# Autodesk Inventor assembly: linac_upper_holder-asm
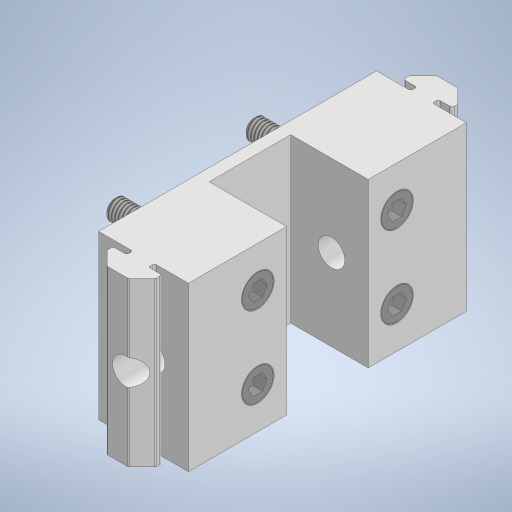
[picture p0: Inventor's stored thumbnail of the model, 512x512]
Saved by Autodesk Inventor 2024 (Build 280153000, 153)
## iProperties
Created: 2025-12-26
Part Number: linac_upper_holder-asm
Document SubType Name: Assembly
Designer: schar
Author: schar
## Documents named in this file (3)
- C:\Users\schar\Desktop\projectBlueprint\AMSTS\hardware\linac_upper_holder-asm.iam
- C:\Users\schar\Desktop\projectBlueprint\AMSTS\hardware\linac_upper_holder.ipt
- C:\Users\schar\Documents\Inventor\Content Center Files\R2024\en-US\ISO 4762(1)\DIN EN ISO 4762 - M5 x 30.ipt
## Components (5 placed, 2 different names)
1. linac_upper_holder:1 — Mate:1, Mate:2, Mate:3, Mate:4, Mate:5, Mate:6, Mate:7, Mate:8
2. DIN EN ISO 4762 M5 x 30:1 — Mate:4, Mate:5
3. DIN EN ISO 4762 M5 x 30:2 — Mate:2, Mate:8
4. DIN EN ISO 4762 M5 x 30:3 — Mate:3, Mate:6
5. DIN EN ISO 4762 M5 x 30:4 — Mate:1, Mate:7
## Relationships (8: Mate 8)
- Mate:1: linac_upper_holder:1 ↔ DIN EN ISO 4762 M5 x 30:4
- Mate:2: linac_upper_holder:1 ↔ DIN EN ISO 4762 M5 x 30:2
- Mate:3: linac_upper_holder:1 ↔ DIN EN ISO 4762 M5 x 30:3
- Mate:4: linac_upper_holder:1 ↔ DIN EN ISO 4762 M5 x 30:1
- Mate:5: linac_upper_holder:1 ↔ DIN EN ISO 4762 M5 x 30:1
- Mate:6: linac_upper_holder:1 ↔ DIN EN ISO 4762 M5 x 30:3
- Mate:7: linac_upper_holder:1 ↔ DIN EN ISO 4762 M5 x 30:4
- Mate:8: linac_upper_holder:1 ↔ DIN EN ISO 4762 M5 x 30:2
